# Autodesk Inventor assembly: B3M-SC-1040-A_ClampHorn
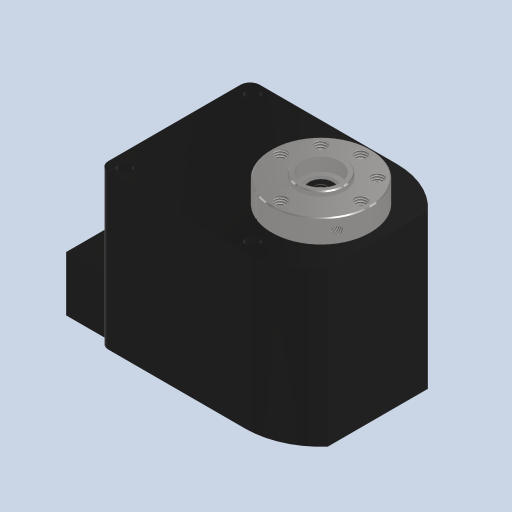
[picture p0: Inventor's stored thumbnail of the model, 512x512]
Saved by Autodesk Inventor 2023 (Build 270158000, 158)
## iProperties
Created: 2024-08-22
Part Number: B3M-SC-1040-A_ClampHorn
Document SubType Name: Assembly
Designer: kiyo
Author: kiyo
## Documents named in this file (3)
- D:\GitHub\inventor\OfficeRobot\ReadyMade\B3M\B3M-SC-1040-A_ClampHorn.iam
- D:\GitHub\inventor\OfficeRobot\ReadyMade\B3M\ClampHorn.ipt
- D:\GitHub\inventor\OfficeRobot\ReadyMade\B3M\B3M-SC-1040-A.ipt
## Components (2 placed, 2 different names)
1. ClampHorn:1 — 挿入:1
2. B3M-SC-1040-A:1 — 挿入:1
## Relationships (1: Insert 1)
- 挿入:1 [Insert] (0.5 mm): ClampHorn:1 ↔ B3M-SC-1040-A:1
